# Autodesk Inventor assembly: Assembly3
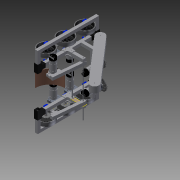
[picture p0: Inventor's stored thumbnail of the model, 180x180]
Saved by Autodesk Inventor 2015 (Build 190159000, 159)
## iProperties
Created: 2014-10-04
Part Number: Assembly3
Document SubType Name: Assembly
Designer: jesse
Author: jesse
## Documents named in this file (34)
- C:\Users\jesse\Desktop\robot\Assembly3.iam
- C:\Users\jesse\Desktop\robot\x base piece.ipt
- C:\Users\jesse\Desktop\robot\y base piece.ipt
- C:\Users\jesse\Desktop\robot\stock parts\am-2648_4inWheel8mmHub\am-2648_4inWheel8mmHub.iam
- C:\Users\jesse\Desktop\robot\stock parts\bronze_bushing_2012\bronze_bushing_2012.ipt
- C:\Users\jesse\Desktop\robot\inside wheel strut.ipt
- C:\Users\jesse\Desktop\robot\set of axle holders.iam
- C:\Users\jesse\Desktop\robot\stock parts\sprocket_25_24t_tetrix_2012\sprocket_25_24t_tetrix_2012.ipt
- C:\Users\jesse\Desktop\robot\stock parts\axle_d-shaft_2012\axle_d-shaft_2012.ipt
- C:\Users\jesse\Desktop\robot\stock parts\tetrix_739376_2pc_motormnt_2013\tetrix_739376_2pc_motormnt_2013-2.iam
- C:\Users\jesse\Desktop\robot\stock parts\am-2964NeveRest\am-2964NeveRest.ipt
- C:\Users\jesse\Desktop\robot\curved piece.ipt
- C:\Users\jesse\Desktop\robot\front peice right.ipt
- C:\Users\jesse\Desktop\robot\front peice left.ipt
- C:\Users\jesse\Desktop\robot\T clamp - bottom.ipt
- C:\Users\jesse\Desktop\robot\T clamp - top.ipt
- C:\Users\jesse\Desktop\robot\roller.ipt
- C:\Users\jesse\Desktop\robot\arm\sidepeices.ipt
- C:\Users\jesse\Desktop\robot\stock parts\dc_motor_mount_2012\dc_motor_mount_2012.ipt
- C:\Users\jesse\Desktop\robot\arm\other side roller axle holder.ipt
- C:\Users\jesse\Desktop\robot\arm\arm axle.ipt
- C:\Users\jesse\Desktop\robot\arm\arm holder mount thing.ipt
- C:\Users\jesse\Desktop\robot\arm\side holders.ipt
- C:\Users\jesse\Desktop\robot\arm\wheel spacers.ipt
- C:\Users\jesse\Desktop\robot\stock parts\hub_motor_shaft_2012\hub_motor_shaft_2012.ipt
- C:\Users\jesse\Desktop\robot\stock parts\axle_set_collar_2012\axle_set_collar_2012.ipt
- C:\Users\jesse\Desktop\robot\stock parts\screw_shcs_6-32_x_1_25_2012\screw_shcs_6-32_x_1_25_2012.ipt
- C:\Users\jesse\Desktop\robot\Part17.ipt
- C:\Users\jesse\Desktop\robot\Part18.ipt
- C:\Users\jesse\Desktop\robot\Conveyor Belt.ipt
- C:\Users\jesse\Desktop\robot\lift\pillar.ipt
- C:\Users\jesse\Desktop\robot\lift\pillar 2.ipt
- C:\Users\jesse\Desktop\robot\lift\Transverse.ipt
- C:\Users\jesse\Desktop\robot\stock parts\gear_80_2011.ipt
## Components (129 placed, 33 different names)
1. x base piece:1 — Angle:7, Angle:8, Angle:9, Flush:34, Flush:35, Mate:73, Flush:38, Flush:113
2. y base piece:2 — Flush:6, Mate:3, Flush:34, Flush:35, Mate:73, Mate:74, Mate:75, Mate:76, Flush:36, Flush:37, Mate:101, Mate:102, Mate:104, Mate:105
3. x base piece:2 — Flush:6, Mate:3, Mate:32, Flush:12, Angle:1, Angle:2, Angle:3, Flush:18, Flush:19, Flush:20, Flush:37, Flush:41, Mate:207
4. am-2648_4inWheel8mmHub:8 [sub-assembly] — Mate:18, Mate:19, Mate:45, Mate:46, Mate:56, Mate:208, Mate:209, Mate:210, Mate:211, Mate:212
5. am-2648_4inWheel8mmHub:9 [sub-assembly] — Mate:20, Mate:21, Mate:43, Mate:44, Mate:57, Mate:213, Mate:214, Mate:215, Mate:216, Mate:217
6. am-2648_4inWheel8mmHub:10 [sub-assembly] — Mate:22, Mate:23, Mate:41, Mate:42, Mate:58, Mate:218, Mate:219, Mate:220, Mate:221, Mate:222
7. am-2648_4inWheel8mmHub:11 [sub-assembly] — Mate:16, Mate:17, Mate:50, Mate:51, Mate:54, Mate:202, Mate:203, Mate:204, Mate:205, Mate:206
8. am-2648_4inWheel8mmHub:12 [sub-assembly] — Mate:12, Mate:47, Mate:52, Mate:55, Mate:186, Mate:189, Mate:190, Mate:191, Mate:192, Mate:193, Mate:194, Mate:195, Mate:196
9. am-2648_4inWheel8mmHub:13 [sub-assembly] — Mate:14, Mate:15, Mate:48, Mate:49, Mate:53, Mate:197, Mate:198, Mate:199, Mate:200, Mate:201
10. bronze_bushing_2012:1 — Mate:12, Mate:186
11. bronze_bushing_2012:2 — Mate:14, Mate:15
12. bronze_bushing_2012:3 — Mate:16, Mate:17
13. bronze_bushing_2012:5 — Mate:20, Mate:21, Mate:34
14. bronze_bushing_2012:6 — Mate:22, Mate:23, Mate:35
15. bronze_bushing_2012:7 — Mate:18, Mate:19, Mate:33
16. inside wheel strut:1 — Mate:40, Flush:14, Angle:4, Angle:5, Angle:6, Mate:67, Mate:68, Flush:26, Flush:27, Angle:12, Angle:13, Mate:75, Flush:40, Mate:98, Mate:103, Flush:58, Mate:135, Mate:136, Angle:14, Mate:147, Mate:149, Mate:152, Mate:207, Mate:238, Flush:109
17. inside wheel strut:2 — Mate:39, Flush:15, Mate:65, Flush:24, Mate:66, Flush:25, Angle:10, Angle:11, Mate:74, Mate:76, Flush:36, Flush:39, Mate:97, Mate:106, Mate:154, Mate:155, Flush:63, Mate:157
18. set of axle holders:1 [sub-assembly] — Flush:13, Flush:16, Flush:21, Flush:22, Flush:23, Mate:188, Mate:234
19. set of axle holders:2 [sub-assembly] — Mate:32, Flush:12, Flush:13, Mate:33, Mate:34, Mate:35, Mate:59, Mate:60, Mate:61, Mate:227, Mate:230, Mate:232
20. set of axle holders:3 [sub-assembly] — Mate:40, Flush:14, Flush:17, Mate:77, Flush:61, Flush:62, Mate:138, Mate:140
21. set of axle holders:4 [sub-assembly] — Mate:39, Flush:15, Flush:16, Flush:17, Mate:62, Mate:63, Mate:64, Mate:142, Mate:144, Mate:146
22. sprocket_25_24t_tetrix_2012:1 — Mate:45, Mate:46, Mate:56, Rotation:4, Mate:88, Mate:89
23. sprocket_25_24t_tetrix_2012:2 — Mate:43, Mate:44, Mate:57, Rotation:3, Rotation:4, Mate:86, Flush:66
24. sprocket_25_24t_tetrix_2012:3 — Mate:41, Mate:42, Mate:58, Rotation:3, Mate:84, Mate:85, Flush:67
25. sprocket_25_24t_tetrix_2012:4 — Mate:47, Mate:52, Mate:55, Rotation:2, Mate:82, Mate:83, Flush:69, Flush:106
26. sprocket_25_24t_tetrix_2012:5 — Mate:48, Mate:49, Mate:53, Rotation:1, Rotation:2, Mate:80, Mate:81, Flush:68, Flush:104, Flush:105
27. sprocket_25_24t_tetrix_2012:6 — Mate:50, Mate:51, Mate:54, Rotation:1, Mate:78, Mate:79, Flush:103
28. axle_d-shaft_2012:1 — Mate:59, Angle:2, Angle:6, Flush:18, Mate:77, Mate:226
29. axle_d-shaft_2012:2 — Mate:64, Flush:21, Angle:7, Mate:141, Mate:233
30. axle_d-shaft_2012:3 — Mate:60, Angle:1, Angle:5, Flush:19, Mate:87, Mate:137, Mate:229
31. axle_d-shaft_2012:4 — Mate:61, Angle:3, Angle:4, Flush:20, Mate:139, Mate:231
32. axle_d-shaft_2012:5 — Mate:62, Angle:9, Flush:23, Mate:145, Mate:187
33. axle_d-shaft_2012:6 — Mate:63, Angle:8, Flush:22, Mate:143
34. tetrix_739376_2pc_motormnt_2013-2:1 [sub-assembly] — Mate:65, Flush:24, Mate:72, Flush:29, Flush:32
35. tetrix_739376_2pc_motormnt_2013-2:2 [sub-assembly] — Mate:66, Flush:25, Mate:69, Flush:28, Flush:33
36. tetrix_739376_2pc_motormnt_2013-2:3 [sub-assembly] — Mate:67, Flush:26, Mate:71, Flush:30, Flush:32
37. tetrix_739376_2pc_motormnt_2013-2:4 [sub-assembly] — Mate:68, Flush:27, Mate:70, Flush:31, Flush:33
38. am-2964NeveRest:1 — Mate:71, Flush:30, Angle:12, Mate:180
39. am-2964NeveRest:2 — Mate:69, Flush:28, Angle:11, Mate:182
40. am-2964NeveRest:3 — Mate:70, Flush:31, Angle:13, Mate:181
41. am-2964NeveRest:4 — Mate:72, Flush:29, Angle:10, Mate:183
42. curved piece:1 — Angle:15, Mate:167, Angle:16, Mate:235
43. front peice right:1 — Flush:38, Flush:39, Mate:95, Mate:96, Flush:113
44. front peice left:1 — Flush:40, Flush:41, Mate:99, Mate:100, Angle:15
45. bronze_bushing_2012:8 — Mate:78, Mate:79
46. bronze_bushing_2012:9 — Mate:80, Mate:81
47. bronze_bushing_2012:10 — Mate:82, Mate:83, Mate:185
48. bronze_bushing_2012:11 — Mate:84, Mate:85, Mate:225
49. bronze_bushing_2012:12 — Mate:86, Mate:87, Mate:224
50. bronze_bushing_2012:13 — Mate:88, Mate:89, Mate:223
51. T clamp - bottom:1 — Flush:42, Mate:91, Flush:43, Mate:96, Mate:97
52. T clamp - top:1 — Flush:42, Mate:91, Flush:43, Mate:95
53. T clamp - bottom:2 — Mate:104, Mate:105, Mate:106
54. T clamp - top:2
55. T clamp - bottom:3 — Mate:98, Mate:100
56. T clamp - top:3 — Mate:99
57. T clamp - bottom:4 — Mate:102
58. T clamp - top:4 — Mate:101, Mate:103
59. roller:1 — Mate:165, Mate:166, Mate:167
60. sidepeices:1 — Mate:160, Mate:163, Mate:164, Flush:65
61. sidepeices:2 — Mate:161, Mate:162, Flush:65, Flush:114
62. dc_motor_mount_2012:1 — Flush:57
63. other side roller axle holder:1 — Mate:165, Flush:114
64. arm axle:1 — Mate:162, Mate:164
65. am-2964NeveRest:6 — Flush:57, Mate:166
66. arm holder mount thing:1 — Flush:58, Mate:135, Mate:148, Mate:150, Mate:151, Mate:161, Flush:107, Flush:108
67. arm holder mount thing:2 — Mate:153, Flush:63, Mate:156, Mate:158, Mate:160, Mate:163
68. side holders:1 — Mate:136, Angle:14, Mate:147, Mate:148, Mate:149
69. wheel spacers:1 — Flush:61, Flush:62, Mate:225
70. wheel spacers:2 — Mate:137, Mate:138, Mate:224
71. wheel spacers:3 — Mate:139, Mate:140, Mate:223
72. wheel spacers:4 — Mate:145, Mate:146, Mate:185
73. wheel spacers:5 — Mate:143, Mate:144
74. wheel spacers:6 — Mate:141, Mate:142
75. side holders:2 — Mate:150, Mate:151, Mate:152
76. side holders:3 — Mate:156, Mate:157, Mate:158
77. side holders:4 — Mate:153, Mate:154, Mate:155
78. hub_motor_shaft_2012:1 — Mate:168, Mate:169, Mate:170, Mate:182
79. sprocket_25_24t_tetrix_2012:7 — Mate:168, Mate:169, Mate:170, Flush:68, Flush:103, Flush:104
80. hub_motor_shaft_2012:2 — Mate:183
81. sprocket_25_24t_tetrix_2012:8 — Flush:69, Flush:105, Flush:106
82. hub_motor_shaft_2012:3 — Mate:180
83. sprocket_25_24t_tetrix_2012:9 — Flush:66
84. hub_motor_shaft_2012:4
85. sprocket_25_24t_tetrix_2012:10 — Mate:181, Flush:67
86. axle_set_collar_2012:1 — Mate:187, Mate:188
87. screw_shcs_6-32_x_1_25_2012:1 — Mate:189, Mate:190
88. screw_shcs_6-32_x_1_25_2012:2 — Mate:191, Mate:192
89. screw_shcs_6-32_x_1_25_2012:3 — Mate:193, Mate:194
90. screw_shcs_6-32_x_1_25_2012:4
91. screw_shcs_6-32_x_1_25_2012:5 — Mate:195, Mate:196
92. screw_shcs_6-32_x_1_25_2012:6 — Flush:71, Mate:199
93. screw_shcs_6-32_x_1_25_2012:7 — Flush:72, Mate:198
94. screw_shcs_6-32_x_1_25_2012:8 — Flush:70, Flush:71, Mate:197, Mate:201
95. screw_shcs_6-32_x_1_25_2012:9 — Flush:70, Flush:72, Mate:200
96. screw_shcs_6-32_x_1_25_2012:14 — Mate:202
97. screw_shcs_6-32_x_1_25_2012:15 — Mate:204, Mate:206
98. screw_shcs_6-32_x_1_25_2012:16 — Mate:205
99. screw_shcs_6-32_x_1_25_2012:17 — Mate:203
100. screw_shcs_6-32_x_1_25_2012:18 — Mate:209, Mate:212
101. screw_shcs_6-32_x_1_25_2012:19 — Mate:210
102. screw_shcs_6-32_x_1_25_2012:20 — Mate:211
103. screw_shcs_6-32_x_1_25_2012:21 — Mate:208
104. screw_shcs_6-32_x_1_25_2012:22 — Mate:213, Mate:217
105. screw_shcs_6-32_x_1_25_2012:23 — Mate:214
106. screw_shcs_6-32_x_1_25_2012:24 — Mate:216
107. screw_shcs_6-32_x_1_25_2012:25 — Mate:215
108. screw_shcs_6-32_x_1_25_2012:26 — Mate:221
109. screw_shcs_6-32_x_1_25_2012:27 — Mate:219, Mate:222
110. screw_shcs_6-32_x_1_25_2012:28 — Mate:220, Mate:228
111. screw_shcs_6-32_x_1_25_2012:29 — Mate:218
112. axle_set_collar_2012:2 — Mate:226, Mate:227, Mate:228
113. axle_set_collar_2012:3 — Mate:229, Mate:230
114. axle_set_collar_2012:4 — Mate:231, Mate:232
115. axle_set_collar_2012:5 — Mate:233, Mate:234
116. Ramp — Angle:16, Mate:235
117. Ramp- support — Flush:107, Flush:108
118. Conveyor Belt:1
119. pillar:1 — Mate:238, Flush:109, Flush:110, Mate:239, Mate:240, Mate:241
120. pillar 2:1 — Flush:110
121. Transverse:1 — Mate:239, Mate:240, Mate:241, Mate:242, Flush:111, Mate:243, Flush:112
122. am-2964NeveRest:7 — Mate:245, Flush:116, Mate:246, Mate:247, Mate:252
123. am-2964NeveRest:8 — Mate:244, Flush:115, Mate:248, Mate:249, Mate:253
124. gear_80_2011:1 — Mate:247, Mate:251
125. gear_80_2011:2 — Mate:248, Mate:250
126. hub_motor_shaft_2012:5 — Mate:246, Mate:251, Mate:252
127. hub_motor_shaft_2012:6 — Mate:249, Mate:250, Mate:253
128. tetrix_739376_2pc_motormnt_2013-2:5 [sub-assembly] — Mate:242, Flush:111, Mate:245, Flush:116
129. tetrix_739376_2pc_motormnt_2013-2:6 [sub-assembly] — Mate:243, Flush:112, Mate:244, Flush:115
## Relationships (322: Mate 207, Flush 95, Angle 16, RelateRotation 4)
- Flush:6: y base piece:2 ↔ x base piece:2
- Mate:3: y base piece:2 ↔ x base piece:2
- [Mate]: x base piece:1 ↔ set of axle holders:1
- [Flush]: x base piece:1 ↔ set of axle holders:1
- [Mate]: am-2648_4inWheel8mmHub:12 ↔ set of axle holders:1
- [Mate]: am-2648_4inWheel8mmHub:13 ↔ set of axle holders:1
- [Mate]: am-2648_4inWheel8mmHub:11 ↔ set of axle holders:1
- Mate:12: am-2648_4inWheel8mmHub:12 ↔ bronze_bushing_2012:1
- Mate:14: am-2648_4inWheel8mmHub:13 ↔ bronze_bushing_2012:2
- Mate:15: am-2648_4inWheel8mmHub:13 ↔ bronze_bushing_2012:2
- Mate:16: am-2648_4inWheel8mmHub:11 ↔ bronze_bushing_2012:3
- Mate:17: am-2648_4inWheel8mmHub:11 ↔ bronze_bushing_2012:3
- Mate:18: am-2648_4inWheel8mmHub:8 ↔ bronze_bushing_2012:7
- Mate:19: am-2648_4inWheel8mmHub:8 ↔ bronze_bushing_2012:7
- Mate:20: am-2648_4inWheel8mmHub:9 ↔ bronze_bushing_2012:5
- Mate:21: am-2648_4inWheel8mmHub:9 ↔ bronze_bushing_2012:5
- Mate:22: am-2648_4inWheel8mmHub:10 ↔ bronze_bushing_2012:6
- Mate:23: am-2648_4inWheel8mmHub:10 ↔ bronze_bushing_2012:6
- Mate:32: x base piece:2 ↔ set of axle holders:2
- Flush:12: x base piece:2 ↔ set of axle holders:2
- Flush:13: set of axle holders:1 ↔ set of axle holders:2
- Mate:33: bronze_bushing_2012:7 ↔ set of axle holders:2
- Mate:34: bronze_bushing_2012:5 ↔ set of axle holders:2
- Mate:35: bronze_bushing_2012:6 ↔ set of axle holders:2
- Mate:39: inside wheel strut:2 ↔ set of axle holders:4
- Mate:40: inside wheel strut:1 ↔ set of axle holders:3
- Flush:14: inside wheel strut:1 ↔ set of axle holders:3
- Flush:15: inside wheel strut:2 ↔ set of axle holders:4
- Flush:16: set of axle holders:1 ↔ set of axle holders:4
- Flush:17: set of axle holders:3 ↔ set of axle holders:4
- Mate:41: am-2648_4inWheel8mmHub:10 ↔ sprocket_25_24t_tetrix_2012:3
- Mate:42: am-2648_4inWheel8mmHub:10 ↔ sprocket_25_24t_tetrix_2012:3
- Mate:43: am-2648_4inWheel8mmHub:9 ↔ sprocket_25_24t_tetrix_2012:2
- Mate:44: am-2648_4inWheel8mmHub:9 ↔ sprocket_25_24t_tetrix_2012:2
- Mate:45: am-2648_4inWheel8mmHub:8 ↔ sprocket_25_24t_tetrix_2012:1
- Mate:46: am-2648_4inWheel8mmHub:8 ↔ sprocket_25_24t_tetrix_2012:1
- Mate:47: am-2648_4inWheel8mmHub:12 ↔ sprocket_25_24t_tetrix_2012:4
- Mate:48: am-2648_4inWheel8mmHub:13 ↔ sprocket_25_24t_tetrix_2012:5
- Mate:49: am-2648_4inWheel8mmHub:13 ↔ sprocket_25_24t_tetrix_2012:5
- Mate:50: am-2648_4inWheel8mmHub:11 ↔ sprocket_25_24t_tetrix_2012:6
- Mate:51: am-2648_4inWheel8mmHub:11 ↔ sprocket_25_24t_tetrix_2012:6
- Mate:52: am-2648_4inWheel8mmHub:12 ↔ sprocket_25_24t_tetrix_2012:4
- Mate:53: am-2648_4inWheel8mmHub:13 ↔ sprocket_25_24t_tetrix_2012:5
- Mate:54: am-2648_4inWheel8mmHub:11 ↔ sprocket_25_24t_tetrix_2012:6
- Mate:55: am-2648_4inWheel8mmHub:12 ↔ sprocket_25_24t_tetrix_2012:4
- Mate:56: am-2648_4inWheel8mmHub:8 ↔ sprocket_25_24t_tetrix_2012:1
- Mate:57: am-2648_4inWheel8mmHub:9 ↔ sprocket_25_24t_tetrix_2012:2
- Mate:58: am-2648_4inWheel8mmHub:10 ↔ sprocket_25_24t_tetrix_2012:3
- Rotation:1 [RelateRotation] (1 ul): sprocket_25_24t_tetrix_2012:5 ↔ sprocket_25_24t_tetrix_2012:6
- Rotation:2 [RelateRotation] (1 ul): sprocket_25_24t_tetrix_2012:4 ↔ sprocket_25_24t_tetrix_2012:5
- Rotation:3 [RelateRotation] (1 ul): sprocket_25_24t_tetrix_2012:2 ↔ sprocket_25_24t_tetrix_2012:3
- Rotation:4 [RelateRotation] (1 ul): sprocket_25_24t_tetrix_2012:1 ↔ sprocket_25_24t_tetrix_2012:2
- Mate:59: set of axle holders:2 ↔ axle_d-shaft_2012:1
- Mate:60: set of axle holders:2 ↔ axle_d-shaft_2012:3
- Mate:61: set of axle holders:2 ↔ axle_d-shaft_2012:4
- Mate:62: set of axle holders:4 ↔ axle_d-shaft_2012:5
- Mate:63: set of axle holders:4 ↔ axle_d-shaft_2012:6
- Mate:64: set of axle holders:4 ↔ axle_d-shaft_2012:2
- Angle:1 (180 deg): x base piece:2 ↔ axle_d-shaft_2012:3
- Angle:2 (180 deg): x base piece:2 ↔ axle_d-shaft_2012:1
- Angle:3 (180 deg): x base piece:2 ↔ axle_d-shaft_2012:4
- Angle:4 (0 deg): inside wheel strut:1 ↔ axle_d-shaft_2012:4
- Angle:5 (0 deg): inside wheel strut:1 ↔ axle_d-shaft_2012:3
- Angle:6 (0 deg): inside wheel strut:1 ↔ axle_d-shaft_2012:1
- Flush:18: x base piece:2 ↔ axle_d-shaft_2012:1
- Flush:19: x base piece:2 ↔ axle_d-shaft_2012:3
- Flush:20: x base piece:2 ↔ axle_d-shaft_2012:4
- Flush:21: set of axle holders:1 ↔ axle_d-shaft_2012:2
- Angle:7 (0 deg): x base piece:1 ↔ axle_d-shaft_2012:2
- Angle:8 (0 deg): x base piece:1 ↔ axle_d-shaft_2012:6
- Angle:9 (0 deg): x base piece:1 ↔ axle_d-shaft_2012:5
- Flush:22: set of axle holders:1 ↔ axle_d-shaft_2012:6
- Flush:23: set of axle holders:1 ↔ axle_d-shaft_2012:5
- Mate:65: inside wheel strut:2 ↔ tetrix_739376_2pc_motormnt_2013-2:1
- Flush:24: inside wheel strut:2 ↔ tetrix_739376_2pc_motormnt_2013-2:1
- Mate:66: inside wheel strut:2 ↔ tetrix_739376_2pc_motormnt_2013-2:2
- Flush:25: inside wheel strut:2 ↔ tetrix_739376_2pc_motormnt_2013-2:2
- Mate:67: inside wheel strut:1 ↔ tetrix_739376_2pc_motormnt_2013-2:3
- Mate:68: inside wheel strut:1 ↔ tetrix_739376_2pc_motormnt_2013-2:4
- Flush:26: inside wheel strut:1 ↔ tetrix_739376_2pc_motormnt_2013-2:3
- Flush:27: inside wheel strut:1 ↔ tetrix_739376_2pc_motormnt_2013-2:4
- Mate:69: tetrix_739376_2pc_motormnt_2013-2:2 ↔ am-2964NeveRest:2
- Mate:70: tetrix_739376_2pc_motormnt_2013-2:4 ↔ am-2964NeveRest:3
- Mate:71: tetrix_739376_2pc_motormnt_2013-2:3 ↔ am-2964NeveRest:1
- Mate:72: tetrix_739376_2pc_motormnt_2013-2:1 ↔ am-2964NeveRest:4
- Flush:28: tetrix_739376_2pc_motormnt_2013-2:2 ↔ am-2964NeveRest:2
- Flush:29: tetrix_739376_2pc_motormnt_2013-2:1 ↔ am-2964NeveRest:4
- Flush:30: tetrix_739376_2pc_motormnt_2013-2:3 ↔ am-2964NeveRest:1
- Flush:31: tetrix_739376_2pc_motormnt_2013-2:4 ↔ am-2964NeveRest:3
- Flush:32: tetrix_739376_2pc_motormnt_2013-2:1 ↔ tetrix_739376_2pc_motormnt_2013-2:3
- Flush:33: tetrix_739376_2pc_motormnt_2013-2:2 ↔ tetrix_739376_2pc_motormnt_2013-2:4
- Angle:10 (90 deg): inside wheel strut:2 ↔ am-2964NeveRest:4
- Angle:11 (90 deg): inside wheel strut:2 ↔ am-2964NeveRest:2
- Angle:12 (-90 deg): inside wheel strut:1 ↔ am-2964NeveRest:1
- Angle:13 (90 deg): inside wheel strut:1 ↔ am-2964NeveRest:3
- Flush:34: x base piece:1 ↔ y base piece:2
- Flush:35: x base piece:1 ↔ y base piece:2
- Mate:73: x base piece:1 ↔ y base piece:2
- Mate:74: y base piece:2 ↔ inside wheel strut:2
- Mate:75: y base piece:2 ↔ inside wheel strut:1
- Mate:76: y base piece:2 ↔ inside wheel strut:2
- Flush:36: y base piece:2 ↔ inside wheel strut:2
- Mate:77: set of axle holders:3 ↔ axle_d-shaft_2012:1
- Flush:37: y base piece:2 ↔ x base piece:2
- Flush:38: x base piece:1 ↔ front peice right:1
- Flush:39: inside wheel strut:2 ↔ front peice right:1
- Flush:40: inside wheel strut:1 ↔ front peice left:1
- Flush:41: x base piece:2 ↔ front peice left:1
- Mate:78: sprocket_25_24t_tetrix_2012:6 ↔ bronze_bushing_2012:8
- Mate:79: sprocket_25_24t_tetrix_2012:6 ↔ bronze_bushing_2012:8
- Mate:80: sprocket_25_24t_tetrix_2012:5 ↔ bronze_bushing_2012:9
- Mate:81: sprocket_25_24t_tetrix_2012:5 ↔ bronze_bushing_2012:9
- Mate:82: sprocket_25_24t_tetrix_2012:4 ↔ bronze_bushing_2012:10
- Mate:83: sprocket_25_24t_tetrix_2012:4 ↔ bronze_bushing_2012:10
- Mate:84: sprocket_25_24t_tetrix_2012:3 ↔ bronze_bushing_2012:11
- Mate:85: sprocket_25_24t_tetrix_2012:3 ↔ bronze_bushing_2012:11
- Mate:86: sprocket_25_24t_tetrix_2012:2 ↔ bronze_bushing_2012:12
- Mate:87: axle_d-shaft_2012:3 ↔ bronze_bushing_2012:12
- Mate:88: sprocket_25_24t_tetrix_2012:1 ↔ bronze_bushing_2012:13
- Mate:89: sprocket_25_24t_tetrix_2012:1 ↔ bronze_bushing_2012:13
- Flush:42: T clamp - bottom:1 ↔ T clamp - top:1
- Mate:91: T clamp - bottom:1 ↔ T clamp - top:1
- Flush:43: T clamp - bottom:1 ↔ T clamp - top:1
- [Flush]: T clamp - bottom:2 ↔ T clamp - top:2
- [Mate]: T clamp - bottom:2 ↔ T clamp - top:2
- [Flush]: T clamp - bottom:2 ↔ T clamp - top:2
- [Flush]: T clamp - bottom:3 ↔ T clamp - top:3
- [Mate]: T clamp - bottom:3 ↔ T clamp - top:3
- [Flush]: T clamp - bottom:3 ↔ T clamp - top:3
- [Flush]: T clamp - bottom:4 ↔ T clamp - top:4
- [Mate]: T clamp - bottom:4 ↔ T clamp - top:4
- [Flush]: T clamp - bottom:4 ↔ T clamp - top:4
- Mate:95: front peice right:1 ↔ T clamp - top:1
- Mate:96: front peice right:1 ↔ T clamp - bottom:1
- Mate:97: inside wheel strut:2 ↔ T clamp - bottom:1
- Mate:98: inside wheel strut:1 ↔ T clamp - bottom:3
- Mate:99: front peice left:1 ↔ T clamp - top:3
- Mate:100: front peice left:1 ↔ T clamp - bottom:3
- Mate:101: y base piece:2 ↔ T clamp - top:4
- Mate:102: y base piece:2 ↔ T clamp - bottom:4
- Mate:103: inside wheel strut:1 ↔ T clamp - top:4
- Mate:104: y base piece:2 ↔ T clamp - bottom:2
- Mate:105: y base piece:2 ↔ T clamp - bottom:2
- Mate:106: inside wheel strut:2 ↔ T clamp - bottom:2
- [Flush]: sidepeices:1 ↔ dc_motor_mount_2012:1
- [Mate]: sidepeices:1 ↔ dc_motor_mount_2012:1
- [Flush]: sidepeices:1 ↔ dc_motor_mount_2012:1
- [Flush]: sidepeices:2 ↔ other side roller axle holder:1
- [Mate]: dc_motor_mount_2012:1 ↔ am-2964NeveRest:6
- [Mate]: sidepeices:2 ↔ other side roller axle holder:1
- [Mate]: arm axle:1 ↔ arm holder mount thing:1
- [Mate]: arm axle:1 ↔ arm holder mount thing:2
- [Flush]: arm holder mount thing:1 ↔ arm holder mount thing:2
- Flush:57: dc_motor_mount_2012:1 ↔ am-2964NeveRest:6
- Flush:58: inside wheel strut:1 ↔ arm holder mount thing:1
- Mate:135: inside wheel strut:1 ↔ arm holder mount thing:1
- Mate:136: inside wheel strut:1 ↔ side holders:1
- Angle:14 (90 deg): inside wheel strut:1 ↔ side holders:1
- Flush:61: set of axle holders:3 ↔ wheel spacers:1
- Flush:62: set of axle holders:3 ↔ wheel spacers:1
- Mate:137: axle_d-shaft_2012:3 ↔ wheel spacers:2
- Mate:138: set of axle holders:3 ↔ wheel spacers:2
- Mate:139: axle_d-shaft_2012:4 ↔ wheel spacers:3
- Mate:140: set of axle holders:3 ↔ wheel spacers:3
- Mate:141: axle_d-shaft_2012:2 ↔ wheel spacers:6
- Mate:142: set of axle holders:4 ↔ wheel spacers:6
- Mate:143: axle_d-shaft_2012:6 ↔ wheel spacers:5
- Mate:144: set of axle holders:4 ↔ wheel spacers:5
- Mate:145: axle_d-shaft_2012:5 ↔ wheel spacers:4
- Mate:146: set of axle holders:4 ↔ wheel spacers:4
- Mate:147: inside wheel strut:1 ↔ side holders:1
- Mate:148: arm holder mount thing:1 ↔ side holders:1
- Mate:149: inside wheel strut:1 ↔ side holders:1
- Mate:150: arm holder mount thing:1 ↔ side holders:2
- Mate:151: arm holder mount thing:1 ↔ side holders:2
- Mate:152: inside wheel strut:1 ↔ side holders:2
- Mate:153: arm holder mount thing:2 ↔ side holders:4
- Mate:154: inside wheel strut:2 ↔ side holders:4
- Mate:155: inside wheel strut:2 ↔ side holders:4
- Flush:63: inside wheel strut:2 ↔ arm holder mount thing:2
- Mate:156: arm holder mount thing:2 ↔ side holders:3
- Mate:157: inside wheel strut:2 ↔ side holders:3
- Mate:158: arm holder mount thing:2 ↔ side holders:3
- Mate:160: sidepeices:1 ↔ arm holder mount thing:2
- Mate:161: sidepeices:2 ↔ arm holder mount thing:1
- Mate:162: sidepeices:2 ↔ arm axle:1
- Mate:163: sidepeices:1 ↔ arm holder mount thing:2
- Mate:164: sidepeices:1 ↔ arm axle:1
- Flush:65: sidepeices:1 ↔ sidepeices:2
- Mate:165: roller:1 ↔ other side roller axle holder:1
- Mate:166: roller:1 ↔ am-2964NeveRest:6
- Angle:15 (0 deg): curved piece:1 ↔ front peice left:1
- Mate:167: curved piece:1 ↔ roller:1
- Mate:168: hub_motor_shaft_2012:1 ↔ sprocket_25_24t_tetrix_2012:7
- Mate:169: hub_motor_shaft_2012:1 ↔ sprocket_25_24t_tetrix_2012:7
- Mate:170: hub_motor_shaft_2012:1 ↔ sprocket_25_24t_tetrix_2012:7
- [Mate]: hub_motor_shaft_2012:2 ↔ sprocket_25_24t_tetrix_2012:8
- [Mate]: hub_motor_shaft_2012:2 ↔ sprocket_25_24t_tetrix_2012:8
- [Mate]: hub_motor_shaft_2012:2 ↔ sprocket_25_24t_tetrix_2012:8
- [Mate]: hub_motor_shaft_2012:3 ↔ sprocket_25_24t_tetrix_2012:9
- [Mate]: hub_motor_shaft_2012:3 ↔ sprocket_25_24t_tetrix_2012:9
- [Mate]: hub_motor_shaft_2012:3 ↔ sprocket_25_24t_tetrix_2012:9
- [Mate]: hub_motor_shaft_2012:4 ↔ sprocket_25_24t_tetrix_2012:10
- [Mate]: hub_motor_shaft_2012:4 ↔ sprocket_25_24t_tetrix_2012:10
- [Mate]: hub_motor_shaft_2012:4 ↔ sprocket_25_24t_tetrix_2012:10
- Mate:180: am-2964NeveRest:1 ↔ hub_motor_shaft_2012:3
- Flush:66: sprocket_25_24t_tetrix_2012:2 ↔ sprocket_25_24t_tetrix_2012:9
- Mate:181: am-2964NeveRest:3 ↔ sprocket_25_24t_tetrix_2012:10
- Flush:67: sprocket_25_24t_tetrix_2012:3 ↔ sprocket_25_24t_tetrix_2012:10
- Mate:182: am-2964NeveRest:2 ↔ hub_motor_shaft_2012:1
- Flush:68: sprocket_25_24t_tetrix_2012:5 ↔ sprocket_25_24t_tetrix_2012:7
- Mate:183: am-2964NeveRest:4 ↔ hub_motor_shaft_2012:2
- Flush:69: sprocket_25_24t_tetrix_2012:4 ↔ sprocket_25_24t_tetrix_2012:8
- Mate:185: bronze_bushing_2012:10 ↔ wheel spacers:4
- Mate:186: am-2648_4inWheel8mmHub:12 ↔ bronze_bushing_2012:1
- Mate:187: axle_d-shaft_2012:5 ↔ axle_set_collar_2012:1
- Mate:188: set of axle holders:1 ↔ axle_set_collar_2012:1
- Mate:189: am-2648_4inWheel8mmHub:12 ↔ screw_shcs_6-32_x_1_25_2012:1
- Mate:190: am-2648_4inWheel8mmHub:12 ↔ screw_shcs_6-32_x_1_25_2012:1
- Mate:191: am-2648_4inWheel8mmHub:12 ↔ screw_shcs_6-32_x_1_25_2012:2
- Mate:192: am-2648_4inWheel8mmHub:12 ↔ screw_shcs_6-32_x_1_25_2012:2
- Mate:193: am-2648_4inWheel8mmHub:12 ↔ screw_shcs_6-32_x_1_25_2012:3
- Mate:194: am-2648_4inWheel8mmHub:12 ↔ screw_shcs_6-32_x_1_25_2012:3
- Mate:195: am-2648_4inWheel8mmHub:12 ↔ screw_shcs_6-32_x_1_25_2012:5
- Mate:196: am-2648_4inWheel8mmHub:12 ↔ screw_shcs_6-32_x_1_25_2012:5
- Flush:70: screw_shcs_6-32_x_1_25_2012:8 ↔ screw_shcs_6-32_x_1_25_2012:9
- Flush:71: screw_shcs_6-32_x_1_25_2012:6 ↔ screw_shcs_6-32_x_1_25_2012:8
- Flush:72: screw_shcs_6-32_x_1_25_2012:7 ↔ screw_shcs_6-32_x_1_25_2012:9
- Mate:197: am-2648_4inWheel8mmHub:13 ↔ screw_shcs_6-32_x_1_25_2012:8
- Mate:198: am-2648_4inWheel8mmHub:13 ↔ screw_shcs_6-32_x_1_25_2012:7
- Mate:199: am-2648_4inWheel8mmHub:13 ↔ screw_shcs_6-32_x_1_25_2012:6
- Mate:200: am-2648_4inWheel8mmHub:13 ↔ screw_shcs_6-32_x_1_25_2012:9
- Mate:201: am-2648_4inWheel8mmHub:13 ↔ screw_shcs_6-32_x_1_25_2012:8
- [Flush]: screw_shcs_6-32_x_1_25_2012:16 ↔ screw_shcs_6-32_x_1_25_2012:17
- [Flush]: screw_shcs_6-32_x_1_25_2012:14 ↔ screw_shcs_6-32_x_1_25_2012:16
- [Flush]: screw_shcs_6-32_x_1_25_2012:15 ↔ screw_shcs_6-32_x_1_25_2012:17
- [Flush]: screw_shcs_6-32_x_1_25_2012:14 ↔ screw_shcs_6-32_x_1_25_2012:17
- [Flush]: screw_shcs_6-32_x_1_25_2012:15 ↔ screw_shcs_6-32_x_1_25_2012:17
- [Flush]: screw_shcs_6-32_x_1_25_2012:14 ↔ screw_shcs_6-32_x_1_25_2012:16
- Mate:202: am-2648_4inWheel8mmHub:11 ↔ screw_shcs_6-32_x_1_25_2012:14
- Mate:203: am-2648_4inWheel8mmHub:11 ↔ screw_shcs_6-32_x_1_25_2012:17
- Mate:204: am-2648_4inWheel8mmHub:11 ↔ screw_shcs_6-32_x_1_25_2012:15
- Mate:205: am-2648_4inWheel8mmHub:11 ↔ screw_shcs_6-32_x_1_25_2012:16
- Mate:206: am-2648_4inWheel8mmHub:11 ↔ screw_shcs_6-32_x_1_25_2012:15
- Mate:207 (76.2 mm): x base piece:2 ↔ inside wheel strut:1
- [Flush]: screw_shcs_6-32_x_1_25_2012:20 ↔ screw_shcs_6-32_x_1_25_2012:21
- [Flush]: screw_shcs_6-32_x_1_25_2012:18 ↔ screw_shcs_6-32_x_1_25_2012:20
- [Flush]: screw_shcs_6-32_x_1_25_2012:19 ↔ screw_shcs_6-32_x_1_25_2012:21
- [Flush]: screw_shcs_6-32_x_1_25_2012:18 ↔ screw_shcs_6-32_x_1_25_2012:21
- [Flush]: screw_shcs_6-32_x_1_25_2012:19 ↔ screw_shcs_6-32_x_1_25_2012:21
- [Flush]: screw_shcs_6-32_x_1_25_2012:18 ↔ screw_shcs_6-32_x_1_25_2012:20
- Mate:208: am-2648_4inWheel8mmHub:8 ↔ screw_shcs_6-32_x_1_25_2012:21
- Mate:209: am-2648_4inWheel8mmHub:8 ↔ screw_shcs_6-32_x_1_25_2012:18
- Mate:210: am-2648_4inWheel8mmHub:8 ↔ screw_shcs_6-32_x_1_25_2012:19
- Mate:211: am-2648_4inWheel8mmHub:8 ↔ screw_shcs_6-32_x_1_25_2012:20
- Mate:212: am-2648_4inWheel8mmHub:8 ↔ screw_shcs_6-32_x_1_25_2012:18
- [Flush]: screw_shcs_6-32_x_1_25_2012:24 ↔ screw_shcs_6-32_x_1_25_2012:25
- [Flush]: screw_shcs_6-32_x_1_25_2012:22 ↔ screw_shcs_6-32_x_1_25_2012:24
- [Flush]: screw_shcs_6-32_x_1_25_2012:23 ↔ screw_shcs_6-32_x_1_25_2012:25
- [Flush]: screw_shcs_6-32_x_1_25_2012:22 ↔ screw_shcs_6-32_x_1_25_2012:25
- [Flush]: screw_shcs_6-32_x_1_25_2012:23 ↔ screw_shcs_6-32_x_1_25_2012:25
- [Flush]: screw_shcs_6-32_x_1_25_2012:22 ↔ screw_shcs_6-32_x_1_25_2012:24
- Mate:213: am-2648_4inWheel8mmHub:9 ↔ screw_shcs_6-32_x_1_25_2012:22
- Mate:214: am-2648_4inWheel8mmHub:9 ↔ screw_shcs_6-32_x_1_25_2012:23
- Mate:215: am-2648_4inWheel8mmHub:9 ↔ screw_shcs_6-32_x_1_25_2012:25
- Mate:216: am-2648_4inWheel8mmHub:9 ↔ screw_shcs_6-32_x_1_25_2012:24
- Mate:217: am-2648_4inWheel8mmHub:9 ↔ screw_shcs_6-32_x_1_25_2012:22
- [Flush]: screw_shcs_6-32_x_1_25_2012:28 ↔ screw_shcs_6-32_x_1_25_2012:29
- [Flush]: screw_shcs_6-32_x_1_25_2012:26 ↔ screw_shcs_6-32_x_1_25_2012:28
- [Flush]: screw_shcs_6-32_x_1_25_2012:27 ↔ screw_shcs_6-32_x_1_25_2012:29
- [Flush]: screw_shcs_6-32_x_1_25_2012:26 ↔ screw_shcs_6-32_x_1_25_2012:29
- [Flush]: screw_shcs_6-32_x_1_25_2012:27 ↔ screw_shcs_6-32_x_1_25_2012:29
- [Flush]: screw_shcs_6-32_x_1_25_2012:26 ↔ screw_shcs_6-32_x_1_25_2012:28
- Mate:218: am-2648_4inWheel8mmHub:10 ↔ screw_shcs_6-32_x_1_25_2012:29
- Mate:219: am-2648_4inWheel8mmHub:10 ↔ screw_shcs_6-32_x_1_25_2012:27
- Mate:220: am-2648_4inWheel8mmHub:10 ↔ screw_shcs_6-32_x_1_25_2012:28
- Mate:221: am-2648_4inWheel8mmHub:10 ↔ screw_shcs_6-32_x_1_25_2012:26
- Mate:222: am-2648_4inWheel8mmHub:10 ↔ screw_shcs_6-32_x_1_25_2012:27
- Mate:223: bronze_bushing_2012:13 ↔ wheel spacers:3
- Mate:224: bronze_bushing_2012:12 ↔ wheel spacers:2
- Mate:225: bronze_bushing_2012:11 ↔ wheel spacers:1
- Mate:226: axle_d-shaft_2012:1 ↔ axle_set_collar_2012:2
- Mate:227: set of axle holders:2 ↔ axle_set_collar_2012:2
- Mate:228: screw_shcs_6-32_x_1_25_2012:28 ↔ axle_set_collar_2012:2
- Mate:229: axle_d-shaft_2012:3 ↔ axle_set_collar_2012:3
- Mate:230: set of axle holders:2 ↔ axle_set_collar_2012:3
- Mate:231: axle_d-shaft_2012:4 ↔ axle_set_collar_2012:4
- Mate:232: set of axle holders:2 ↔ axle_set_collar_2012:4
- Mate:233: axle_d-shaft_2012:2 ↔ axle_set_collar_2012:5
- Mate:234: set of axle holders:1 ↔ axle_set_collar_2012:5
- Flush:103: sprocket_25_24t_tetrix_2012:6 ↔ sprocket_25_24t_tetrix_2012:7
- Flush:104: sprocket_25_24t_tetrix_2012:5 ↔ sprocket_25_24t_tetrix_2012:7
- Flush:105: sprocket_25_24t_tetrix_2012:5 ↔ sprocket_25_24t_tetrix_2012:8
- Flush:106: sprocket_25_24t_tetrix_2012:4 ↔ sprocket_25_24t_tetrix_2012:8
- Angle:16 (85 deg): curved piece:1 ↔ Ramp
- Mate:235: curved piece:1 ↔ Ramp
- Flush:107: arm holder mount thing:1 ↔ Ramp- support
- Flush:108: arm holder mount thing:1 ↔ Ramp- support
- Mate:238: inside wheel strut:1 ↔ pillar:1
- Flush:109: inside wheel strut:1 ↔ pillar:1
- Flush:110: pillar:1 ↔ pillar 2:1
- Mate:239: pillar:1 ↔ Transverse:1
- Mate:240: pillar:1 ↔ Transverse:1
- Mate:241: pillar:1 ↔ Transverse:1
- Mate:242: Transverse:1 ↔ tetrix_739376_2pc_motormnt_2013-2:5
- Flush:111: Transverse:1 ↔ tetrix_739376_2pc_motormnt_2013-2:5
- Mate:243: Transverse:1 ↔ tetrix_739376_2pc_motormnt_2013-2:6
- Flush:112: Transverse:1 ↔ tetrix_739376_2pc_motormnt_2013-2:6
- Flush:113: x base piece:1 ↔ front peice right:1
- Flush:114 (9.144 mm): sidepeices:2 ↔ other side roller axle holder:1
- Mate:244: am-2964NeveRest:8 ↔ tetrix_739376_2pc_motormnt_2013-2:6
- Flush:115: am-2964NeveRest:8 ↔ tetrix_739376_2pc_motormnt_2013-2:6
- Mate:245: am-2964NeveRest:7 ↔ tetrix_739376_2pc_motormnt_2013-2:5
- Flush:116: am-2964NeveRest:7 ↔ tetrix_739376_2pc_motormnt_2013-2:5
- Mate:246: am-2964NeveRest:7 ↔ hub_motor_shaft_2012:5
- Mate:247: am-2964NeveRest:7 ↔ gear_80_2011:1
- Mate:248: am-2964NeveRest:8 ↔ gear_80_2011:2
- Mate:249: am-2964NeveRest:8 ↔ hub_motor_shaft_2012:6
- Mate:250: gear_80_2011:2 ↔ hub_motor_shaft_2012:6
- Mate:251: gear_80_2011:1 ↔ hub_motor_shaft_2012:5
- Mate:252 (2.54 mm): am-2964NeveRest:7 ↔ hub_motor_shaft_2012:5
- Mate:253 (2.54 mm): am-2964NeveRest:8 ↔ hub_motor_shaft_2012:6
## Named parameters: d171_d168 = 0 mm, d172_d169 = 0 mm, d173_d170 = 0 mm, d174_d168 = 0 mm, d175_d169 = 0 mm, d176_d170 = 0 mm, d177_d168 = 0 mm, d178_d169 = 0 mm, d179_d170 = 0 mm, d225_d26 = 0 mm, d226_d27 = 0 mm, d228_d29 = 0 mm, d230_d31 = 0 mm, d288_d285 = 0 mm, d289_d286 = 0 mm, d290_d287 = 0 mm, d291_d285 = 0 mm, d292_d286 = 0 mm, d293_d287 = 0 mm, d294_d285 = 0 mm, d295_d286 = 0 mm, d296_d287 = 0 mm, d340_d334_d326 = 0 mm, d341_d335_d327 = 0 mm, d342_d336_d328 = 0 mm, d343_d337 = 0 mm, d344_d338 = 0 mm, d345_d339 = 0 mm, d352_d334_d326 = 0 mm, d353_d335_d327 = 0 mm, d354_d336_d328 = 0 mm, d355_d337 = 0 mm, d356_d338 = 0 mm, d357_d339 = 0 mm, d363_d334_d326 = 0 mm, d364_d335_d327 = 0 mm, d365_d336_d328 = 0 mm, d366_d337 = 0 mm, d367_d338 = 0 mm, d368_d339 = 0 mm, d374_d334_d326 = 0 mm, d375_d335_d327 = 0 mm, d376_d336_d328 = 0 mm, d377_d337 = 0 mm, d378_d338 = 0 mm, d379_d339 = 0 mm
